# Autodesk Inventor assembly: assy-link1
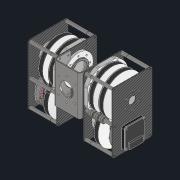
[picture p0: Inventor's stored thumbnail of the model, 180x180]
Saved by Autodesk Inventor 2022 (Build 260153000, 153)
## iProperties
Created: 2021-09-17
Part Number: assy-link1
Document SubType Name: Assembly
Designer: Yuta Kage
Author: Yuta Kage
## Documents named in this file (7)
- C:\Users\yuta0\Documents\GitHub\catchrobo_hardware\model_v2\assy-link1.iam
- C:\Users\yuta0\Documents\GitHub\catchrobo_hardware\model_v2\steelplate2.ipt
- C:\Users\yuta0\Documents\GitHub\catchrobo_hardware\model_v2\unit.iam
- C:\Users\yuta0\Documents\GitHub\catchrobo_hardware\model_v2\base8.ipt
- C:\Users\yuta0\Documents\GitHub\catchrobo_hardware\assy-robot\B6808ZZ.ipt
- C:\Users\yuta0\Documents\GitHub\catchrobo_hardware\model_v2\base9.ipt
- C:\Users\yuta0\Documents\Tokyo Robotics\torobo_3axface\B6811ZZ.ipt
## Components (7 placed, 6 different names)
1. steelplate2:1 — メイト:8, メイト:9, メイト:10, メイト:11, メイト:12, メイト:13
2. unit:4 [sub-assembly] — メイト:8, メイト:9, メイト:10, メイト:19, メイト:20
3. unit:5 [sub-assembly] — メイト:11, メイト:12, メイト:13, メイト:14, メイト:15, メイト:16
4. base8:1 — メイト:14, メイト:15, メイト:16, メイト:17, メイト:18
5. B6808ZZ:1 — メイト:17, メイト:18
6. base9:1 — メイト:19, メイト:20, メイト:21, メイト:22
7. B6811ZZ:1 — メイト:21, メイト:22
## Relationships (15: Mate 15)
- メイト:8 [Mate]: steelplate2:1 ↔ unit:4
- メイト:9 [Mate]: steelplate2:1 ↔ unit:4
- メイト:10 [Mate]: steelplate2:1 ↔ unit:4
- メイト:11 [Mate]: steelplate2:1 ↔ unit:5
- メイト:12 [Mate]: steelplate2:1 ↔ unit:5
- メイト:13 [Mate]: steelplate2:1 ↔ unit:5
- メイト:14 [Mate]: unit:5 ↔ base8:1
- メイト:15 [Mate]: unit:5 ↔ base8:1
- メイト:16 [Mate]: unit:5 ↔ base8:1
- メイト:17 [Mate]: base8:1 ↔ B6808ZZ:1
- メイト:18 [Mate]: base8:1 ↔ B6808ZZ:1
- メイト:19 [Mate]: unit:4 ↔ base9:1
- メイト:20 [Mate]: unit:4 ↔ base9:1
- メイト:21 [Mate]: base9:1 ↔ B6811ZZ:1
- メイト:22 [Mate]: base9:1 ↔ B6811ZZ:1
